# Autodesk Inventor assembly: sail
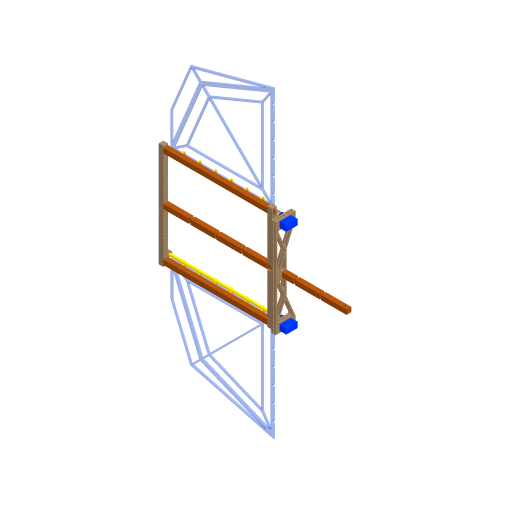
[picture p0: Inventor's stored thumbnail of the model, 512x512]
Saved by Autodesk Inventor 2024 (Build 280153000, 153)
## iProperties
Created: 2024-04-09
Document SubType Name: Assembly
Designer: USER
Mass: 217.661 g
Surface Area: 2188.23 cm^2
Volume: 217.661 cm^3
Density: 1 g/cm^3
Author: 第26組
Title: sail
## Documents named in this file (13)
- C:\Users\op04o\OneDrive\桌面\實務\final\圖檔\DesignVer2_encoder_MG996\sail.iam
- C:\Users\op04o\OneDrive\桌面\實務\final\圖檔\DesignVer2_encoder_MG996\main_Bar.ipt
- C:\Users\op04o\OneDrive\桌面\實務\final\圖檔\DesignVer2_encoder_MG996\main_Bar_3.ipt
- C:\Users\op04o\OneDrive\桌面\實務\final\圖檔\DesignVer2_encoder_MG996\Lower_Bar.ipt
- C:\Users\op04o\OneDrive\桌面\實務\final\圖檔\DesignVer2_encoder_MG996\upper_Bar.ipt
- C:\Users\op04o\OneDrive\桌面\實務\final\圖檔\DesignVer2_encoder_MG996\upper_Bar_3.ipt
- C:\Users\op04o\OneDrive\桌面\實務\final\圖檔\DesignVer2_encoder_MG996\side_Bar.ipt
- C:\Users\op04o\OneDrive\桌面\實務\final\圖檔\DesignVer2_encoder_MG996\[3DP]bar.ipt
- C:\Users\op04o\OneDrive\桌面\實務\final\圖檔\DesignVer2_encoder_MG996\Servo Motor SG90.ipt
- C:\Users\op04o\OneDrive\桌面\實務\final\圖檔\DesignVer2_encoder_MG996\side_motor.ipt
- C:\Users\op04o\OneDrive\桌面\實務\final\圖檔\DesignVer2_encoder_MG996\side_sail.ipt
- C:\Users\op04o\OneDrive\桌面\實務\final\圖檔\DesignVer2_encoder_MG996\[3DP]double_bar.ipt
- C:\Users\op04o\OneDrive\桌面\實務\final\圖檔\DesignVer2_encoder_MG996\side_sail_2.ipt
## Components (27 placed, 12 different names)
1. main_Bar:1 — Flush:1, Flush:2, Mate:2, Mate:7, Mate:11
2. main_Bar:2 — Flush:1, Flush:2, Flush:3, Flush:4, Mate:1, Mate:2, Mate:5, Mate:6
3. main_Bar_3:1 — Flush:3, Flush:4, Mate:1, Mate:10, Flush:13
4. Lower_Bar:1 — Flush:5, Mate:4, Flush:8, Angle:1
5. Lower_Bar:2 — Flush:5, Flush:6, Mate:3, Mate:4, Flush:7, Flush:8, Mate:28
6. upper_Bar:1 — Mate:9, Flush:10, Flush:11, Mate:10, Mate:26
7. upper_Bar:2 — Mate:8, Mate:9, Flush:9, Flush:10, Flush:11, Flush:12, Flush:13
8. upper_Bar_3:1 — Mate:8, Flush:9, Flush:12, Mate:11, Mate:25, Mate:27
9. Lower_Bar:3 — Flush:6, Mate:3, Flush:7, Mate:5, Mate:6, Mate:7, Mate:16, Mate:17, Mate:18, Mate:19, Mate:20, Mate:21, Angle:2
10. side_Bar:1 — Mate:12, Flush:14, Flush:17, Mate:21, Angle:6
11. side_Bar:2 — Mate:12, Mate:13, Flush:14, Flush:15, Flush:16, Flush:17, Mate:20
12. side_Bar:3 — Mate:13, Flush:15, Flush:16, Mate:19
13. side_Bar:4 — Flush:18, Flush:20, Mate:14
14. side_Bar:5 — Flush:18, Flush:19, Flush:20, Flush:21, Mate:14, Mate:15, Mate:16, Mate:18
15. side_Bar:6 — Flush:19, Flush:21, Mate:15, Mate:17, Angle:5
16. [3DP]bar:1 — Mate:24, Mate:25, Mate:26, Mate:29, Mate:36, Mate:37, Mate:38
17. [3DP]bar:2 — Mate:27, Mate:28, Mate:30, Mate:31, Mate:39, Mate:40, Mate:41
18. Servo Motor SG90:1 — Mate:30, Mate:31, Angle:2, Mate:32, Mate:33, Mate:34, Mate:35
19. Servo Motor SG90:2 — Mate:24, Mate:29, Angle:1
20. side_motor:1 — Mate:32, Mate:33, Mate:34, Flush:22, Flush:23
21. side_motor:2 — Flush:22, Flush:23, Mate:35
22. side_sail:1 — Mate:36, Mate:37, Mate:38, Mate:45, Mate:46, Angle:6, Angle:8
23. side_sail:2 — Mate:39, Mate:40, Mate:41, Mate:42, Angle:4, Mate:43, Flush:24, Angle:5, Angle:7
24. [3DP]double_bar:1 — Mate:45, Mate:46, Mate:47, Mate:48
25. [3DP]double_bar:2 — Mate:42, Angle:4, Mate:43, Mate:44
26. side_sail_2:1 — Flush:24, Mate:44, Angle:7
27. side_sail_2:2 — Mate:47, Mate:48, Angle:8
## Relationships (77: Mate 46, Flush 24, Angle 7)
- Flush:1: main_Bar:1 ↔ main_Bar:2
- Flush:2: main_Bar:1 ↔ main_Bar:2
- Flush:3: main_Bar:2 ↔ main_Bar_3:1
- Flush:4: main_Bar:2 ↔ main_Bar_3:1
- Mate:1: main_Bar:2 ↔ main_Bar_3:1
- Mate:2: main_Bar:1 ↔ main_Bar:2
- Flush:5: Lower_Bar:1 ↔ Lower_Bar:2
- Flush:6: Lower_Bar:2 ↔ Lower_Bar:3
- Mate:3: Lower_Bar:2 ↔ Lower_Bar:3
- Mate:4: Lower_Bar:1 ↔ Lower_Bar:2
- Flush:7: Lower_Bar:2 ↔ Lower_Bar:3
- Flush:8: Lower_Bar:1 ↔ Lower_Bar:2
- Mate:5: main_Bar:2 ↔ Lower_Bar:3
- Mate:6: main_Bar:2 ↔ Lower_Bar:3
- Mate:7: main_Bar:1 ↔ Lower_Bar:3
- Mate:8: upper_Bar:2 ↔ upper_Bar_3:1
- Mate:9: upper_Bar:1 ↔ upper_Bar:2
- Flush:9: upper_Bar:2 ↔ upper_Bar_3:1
- Flush:10: upper_Bar:1 ↔ upper_Bar:2
- Flush:11: upper_Bar:1 ↔ upper_Bar:2
- Flush:12: upper_Bar:2 ↔ upper_Bar_3:1
- Mate:10: main_Bar_3:1 ↔ upper_Bar:1
- Flush:13: main_Bar_3:1 ↔ upper_Bar:2
- Mate:11: main_Bar:1 ↔ upper_Bar_3:1
- Mate:12: side_Bar:1 ↔ side_Bar:2
- Mate:13: side_Bar:2 ↔ side_Bar:3
- Flush:14: side_Bar:1 ↔ side_Bar:2
- Flush:15: side_Bar:2 ↔ side_Bar:3
- Flush:16: side_Bar:2 ↔ side_Bar:3
- Flush:17: side_Bar:1 ↔ side_Bar:2
- Flush:18: side_Bar:4 ↔ side_Bar:5
- Flush:19: side_Bar:5 ↔ side_Bar:6
- Flush:20: side_Bar:4 ↔ side_Bar:5
- Flush:21: side_Bar:5 ↔ side_Bar:6
- Mate:14: side_Bar:4 ↔ side_Bar:5
- Mate:15: side_Bar:5 ↔ side_Bar:6
- Mate:16: Lower_Bar:3 ↔ side_Bar:5
- Mate:17: Lower_Bar:3 ↔ side_Bar:6
- Mate:18: Lower_Bar:3 ↔ side_Bar:5
- Mate:19: Lower_Bar:3 ↔ side_Bar:3
- Mate:20: Lower_Bar:3 ↔ side_Bar:2
- Mate:21: Lower_Bar:3 ↔ side_Bar:1
- Mate:24: [3DP]bar:1 ↔ Servo Motor SG90:2
- Mate:25: upper_Bar_3:1 ↔ [3DP]bar:1
- Mate:26: upper_Bar:1 ↔ [3DP]bar:1
- Mate:27: upper_Bar_3:1 ↔ [3DP]bar:2
- Mate:28: Lower_Bar:2 ↔ [3DP]bar:2
- Mate:29: [3DP]bar:1 ↔ Servo Motor SG90:2
- Mate:30: [3DP]bar:2 ↔ Servo Motor SG90:1
- Mate:31: [3DP]bar:2 ↔ Servo Motor SG90:1
- Angle:1 (0 deg): Lower_Bar:1 ↔ Servo Motor SG90:2
- Angle:2 (0 deg): Lower_Bar:3 ↔ Servo Motor SG90:1
- Mate:32: Servo Motor SG90:1 ↔ side_motor:1
- Mate:33: Servo Motor SG90:1 ↔ side_motor:1
- Mate:34: Servo Motor SG90:1 ↔ side_motor:1
- Flush:22: side_motor:1 ↔ side_motor:2
- Flush:23: side_motor:1 ↔ side_motor:2
- Mate:35: Servo Motor SG90:1 ↔ side_motor:2
- Mate:36: [3DP]bar:1 ↔ side_sail:1
- Mate:37: [3DP]bar:1 ↔ side_sail:1
- Mate:38: [3DP]bar:1 ↔ side_sail:1
- Mate:39: [3DP]bar:2 ↔ side_sail:2
- Mate:40: [3DP]bar:2 ↔ side_sail:2
- Mate:41: [3DP]bar:2 ↔ side_sail:2
- Mate:42: side_sail:2 ↔ [3DP]double_bar:2
- Angle:4 (0 deg): side_sail:2 ↔ [3DP]double_bar:2
- Mate:43: side_sail:2 ↔ [3DP]double_bar:2
- Flush:24: side_sail:2 ↔ side_sail_2:1
- Mate:44: [3DP]double_bar:2 ↔ side_sail_2:1
- Mate:45: side_sail:1 ↔ [3DP]double_bar:1
- Mate:46: side_sail:1 ↔ [3DP]double_bar:1
- Mate:47: [3DP]double_bar:1 ↔ side_sail_2:2
- Mate:48: [3DP]double_bar:1 ↔ side_sail_2:2
- Angle:5 (90 deg): side_Bar:6 ↔ side_sail:2
- Angle:6 (90 deg): side_Bar:1 ↔ side_sail:1
- Angle:7 (0 deg): side_sail:2 ↔ side_sail_2:1
- Angle:8 (0 deg): side_sail:1 ↔ side_sail_2:2
